# Autodesk Inventor assembly: FXR_HipServo
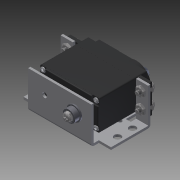
[picture p0: Inventor's stored thumbnail of the model, 180x180]
Saved by Autodesk Inventor 2015 (Build 190159000, 159)
## iProperties
Created: 2015-05-21
Part Number: FXR_HipServo
Document SubType Name: Assembly
Designer: Quinn
Author: Quinn
## Documents named in this file (7)
- C:\Users\Quinn\Desktop\3DCNC Design\InventorModels\Assemblies\FXR_HipServo.iam
- C:\Users\Quinn\Desktop\3DCNC Design\InventorModels\Metal\Brackets\asb-04-ServoMount.ipt
- C:\Users\Quinn\Desktop\3DCNC Design\InventorModels\Electronics\Servo\standard_servo.iam
- C:\Users\Quinn\Desktop\3DCNC Design\InventorModels\Assemblies\FL_Servo_Bracket\Design Accelerator\Bolted Connection3.iam
- C:\Users\Quinn\Desktop\3DCNC Design\InventorModels\Assemblies\FL_Servo_Bracket\Design Accelerator\Bolted Connection4.iam
- C:\Users\Quinn\Desktop\3DCNC Design\InventorModels\Hardware\Bearings\BB-03.ipt
- C:\Users\Quinn\Desktop\3DCNC Design\InventorModels\Assemblies\FXR_HipServo\Design Accelerator\Bolted Connection1.iam
## Components (6 placed, 4 different names)
1. asb-04-ServoMount:1 — Mate:1, Insert:1
2. standard_servo:1 [sub-assembly] — Mate:1, Mate:2, Mate:3, Mate:4, Mate:5
3. Bolted Connection:1 [sub-assembly] — Mate:2, Mate:3
4. Bolted Connection:2 [sub-assembly] — Mate:4, Mate:5
5. BB-03:1 — Insert:1, Mate:6, Mate:7
6. Bolted Connection:3 [sub-assembly] — Mate:6, Mate:7
## Relationships (8: Mate 7, Insert 1)
- Mate:1: asb-04-ServoMount:1 ↔ standard_servo:1
- Mate:2: standard_servo:1 ↔ Bolted Connection:1
- Mate:3: standard_servo:1 ↔ Bolted Connection:1
- Mate:4: standard_servo:1 ↔ Bolted Connection:2
- Mate:5: standard_servo:1 ↔ Bolted Connection:2
- Insert:1: asb-04-ServoMount:1 ↔ BB-03:1
- Mate:6: BB-03:1 ↔ Bolted Connection:3
- Mate:7: BB-03:1 ↔ Bolted Connection:3
